# Autodesk Inventor assembly: 1-104
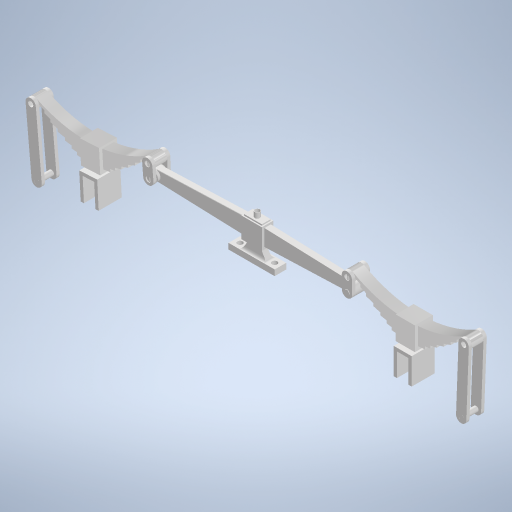
[picture p0: Inventor's stored thumbnail of the model, 512x512]
Saved by Autodesk Inventor 2024.2 (Build 282272000, 272)
## iProperties
Created: 2024-11-02
Part Number: 1-104
Document SubType Name: Assembly
Designer: Jimena Brenes
Author: Jimena Brenes
## Documents named in this file (4)
- C:\Users\Jimena Brenes\OneDrive\Escritorio\1-104\1-104.iam
- C:\Users\Jimena Brenes\OneDrive\Escritorio\1-102\102.iam
- C:\Users\Jimena Brenes\OneDrive\Escritorio\locomotora\HUDSON-1-12-AXLE BROX SPRING.ipt
- C:\Users\Jimena Brenes\OneDrive\Escritorio\locomotora\HUDSON-1-13 LEAFSPING SOLID EQUALISER.ipt
## Components (4 placed, 3 different names)
1. 102:1 [sub-assembly] — Mate:2
2. HUDSON-1-12-AXLE BROX SPRING:1 — Mate:1, Mate:2, Mate:3, Mate:4
3. HUDSON-1-13 LEAFSPING SOLID EQUALISER:1 — Mate:3, Mate:4
4. 102:2 [sub-assembly] — Mate:1
## Relationships (4: Mate 4)
- Mate:1: HUDSON-1-12-AXLE BROX SPRING:1 ↔ 102:2
- Mate:2: 102:1 ↔ HUDSON-1-12-AXLE BROX SPRING:1
- Mate:3: HUDSON-1-12-AXLE BROX SPRING:1 ↔ HUDSON-1-13 LEAFSPING SOLID EQUALISER:1
- Mate:4: HUDSON-1-12-AXLE BROX SPRING:1 ↔ HUDSON-1-13 LEAFSPING SOLID EQUALISER:1
